# Autodesk Inventor assembly: SuspensionAssembly
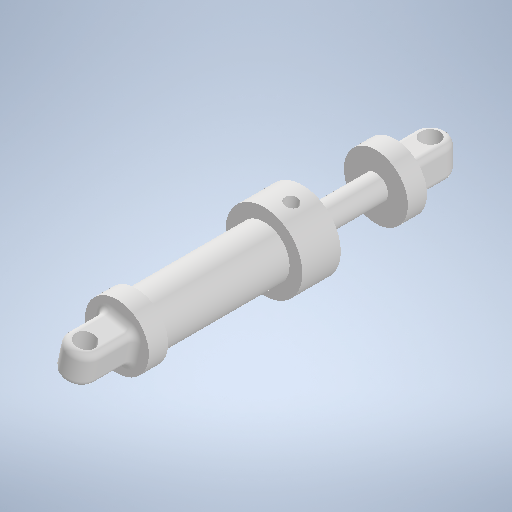
[picture p0: Inventor's stored thumbnail of the model, 512x512]
Saved by Autodesk Inventor 2025.2 (Build 292293000, 293)
## iProperties
Created: 2025-01-06
Part Number: SuspensionAssembly
Document SubType Name: Assembly
Designer: SEON
Author: SEON
## Documents named in this file (4)
- C:\Users\SEON\Documents\Inventor\ProjectRAI\SuspensionAssembly.iam
- C:\Users\SEON\Documents\Inventor\ProjectRAI\SuspensionBase.ipt
- C:\Users\SEON\Documents\Inventor\ProjectRAI\SuspensionCap.ipt
- C:\Users\SEON\Documents\Inventor\ProjectRAI\SuspensionLock.ipt
## Components (4 placed, 3 different names)
1. SuspensionBase:1 — 메이트:1, 메이트:2, 메이트:3, 메이트:4, 메이트:5, 메이트:12
2. SuspensionCap:1 — 메이트:4, 메이트:5, 메이트:6, 메이트:7, 메이트:8, 메이트:9, 메이트:10, 메이트:11
3. SuspensionLock:1 — 메이트:6, 메이트:7, 메이트:8
4. SuspensionLock:2 — 메이트:9, 메이트:10, 메이트:11, 메이트:12
## Relationships (12: Mate 12)
- 메이트:1 [Mate]: SuspensionBase:1
- 메이트:2 [Mate]: SuspensionBase:1
- 메이트:3 [Mate]: SuspensionBase:1
- 메이트:4 [Mate]: SuspensionBase:1 ↔ SuspensionCap:1
- 메이트:5 [Mate]: SuspensionBase:1 ↔ SuspensionCap:1
- 메이트:6 [Mate]: SuspensionCap:1 ↔ SuspensionLock:1
- 메이트:7 [Mate]: SuspensionCap:1 ↔ SuspensionLock:1
- 메이트:8 [Mate]: SuspensionCap:1 ↔ SuspensionLock:1
- 메이트:9 [Mate]: SuspensionCap:1 ↔ SuspensionLock:2
- 메이트:10 [Mate]: SuspensionCap:1 ↔ SuspensionLock:2
- 메이트:11 [Mate]: SuspensionCap:1 ↔ SuspensionLock:2
- 메이트:12 [Mate]: SuspensionBase:1 ↔ SuspensionLock:2
